# Autodesk Inventor assembly: rplidar
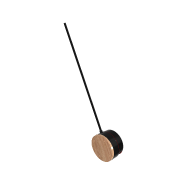
[picture p0: Inventor's stored thumbnail of the model, 180x180]
Saved by Autodesk Inventor 2020.3 (Build 243373000, 373)
## iProperties
Created: 2020-09-30
Part Number: rplidar
Document SubType Name: Assembly
Designer: Svend
Author: Svend
## Documents named in this file (4)
- C:\Users\Svend\OneDrive\Documents\GitHub\Rolstoel\rplidar.iam
- C:\Users\Svend\OneDrive\Documents\GitHub\Rolstoel\onderkant rplidar.ipt
- C:\Users\Svend\OneDrive\Documents\GitHub\Rolstoel\bovenkant rplidar.ipt
- C:\Users\Svend\OneDrive\Documents\GitHub\Rolstoel\spacer lidar.ipt
## Components (3 placed, 3 different names)
1. onderkant rplidar:1 — Mate:1, Mate:2, Mate:3, Flush:1, Flush:2
2. bovenkant rplidar:1 — Mate:1, Mate:2, Mate:3
3. spacer lidar:1 — Flush:1, Flush:2
## Relationships (5: Mate 3, Flush 2)
- Mate:1: onderkant rplidar:1 ↔ bovenkant rplidar:1
- Mate:2 (1 mm): onderkant rplidar:1 ↔ bovenkant rplidar:1
- Mate:3: onderkant rplidar:1 ↔ bovenkant rplidar:1
- Flush:1: onderkant rplidar:1 ↔ spacer lidar:1
- Flush:2: onderkant rplidar:1 ↔ spacer lidar:1
